# Autodesk Inventor assembly: ASSY,ROBOT,2026
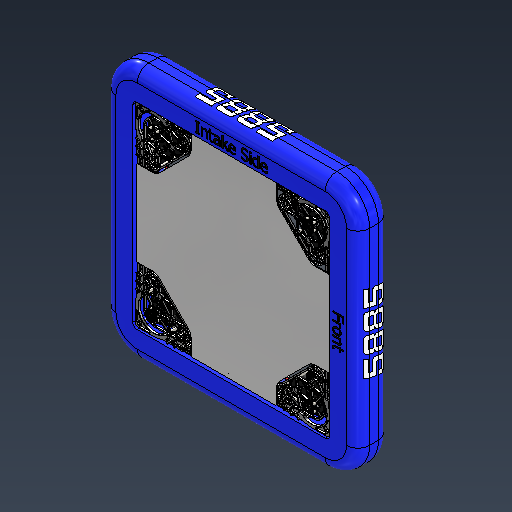
[picture p0: Inventor's stored thumbnail of the model, 512x512]
Saved by Autodesk Inventor 2026 (Build 300175050, 175E)
## iProperties
Created: 2026-01-24
Part Number: ASSY,ROBOT,2026
Document SubType Name: Assembly
Designer: Jthib
Mass: 30551.5 g
Surface Area: 51635 cm^2
Volume: 39972.2 cm^3
Density: 0.764319 g/cm^3
Author: Jthib
## Documents named in this file (3)
- C:\Users\Jthib\Documents\GitHub\2026-Robot-Mechanical\ASSY,ROBOT,2026.iam
- C:\Users\Jthib\Documents\GitHub\2026-Robot-Mechanical\Chassis\CHASSIS.iam
- C:\Users\Jthib\Documents\GitHub\2026-Robot-Mechanical\Chassis\Bumpers.ipt
## Components (2 placed, 2 different names)
1. CHASSIS:1 [sub-assembly] — Flush:1, Flush:2, Flush:3, Flush:4
2. Bumpers:1 — Flush:4, Flush:5, Flush:6
## Relationships (6: Flush 6)
- Flush:1 (-349.25 mm): CHASSIS:1
- Flush:2 (349.25 mm): CHASSIS:1
- Flush:3: CHASSIS:1
- Flush:4 (-12.7 mm): CHASSIS:1 ↔ Bumpers:1
- Flush:5: Bumpers:1
- Flush:6: Bumpers:1
